# Autodesk Inventor assembly: 2013 Drive in a Day Frame
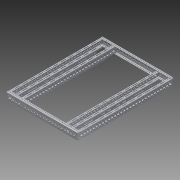
[picture p0: Inventor's stored thumbnail of the model, 180x180]
Saved by Autodesk Inventor 2013 (Build 170138000, 138)
## iProperties
Created: 2013-05-24
Part Number: 2013 Drive in a Day Frame
Document SubType Name: Assembly
Designer: natsidhu
Author: natsidhu
## Documents named in this file (3)
- \\lmss\students\Robotics\CAD Files\COTS Parts\Kit Frame - VexPro\2013 Drive in a Day Frame.iam
- \\lmss\students\Robotics\CAD Files\COTS Parts\Kit Frame - VexPro\217-2593-002 Rev3 - Front Rail.ipt
- \\lmss\students\Robotics\CAD Files\COTS Parts\Kit Frame - VexPro\217-2593-001 Rev2 - Side Rail.ipt
## Components (6 placed, 2 different names)
1. 217-2593-002 Rev3 - Front Rail:1 — Flush:1, Mate:2, Flush:2, Mate:9, Flush:5, Mate:11, Flush:6
2. 217-2593-001 Rev2 - Side Rail:1 — Mate:1, Mate:2, Mate:4, Mate:5, Mate:7, Flush:2, Flush:3
3. 217-2593-001 Rev2 - Side Rail:2 — Mate:8, Mate:9, Flush:4
4. 217-2593-002 Rev3 - Front Rail:2 — Mate:5, Mate:7, Flush:3, Mate:8, Flush:4, Mate:12
5. 217-2593-001 Rev2 - Side Rail:3 — Flush:6, Flush:7, Mate:12
6. 217-2593-001 Rev2 - Side Rail:4 — Flush:5, Mate:10, Mate:11
## Relationships (17: Mate 10, Flush 7)
- Flush:1: 217-2593-002 Rev3 - Front Rail:1
- Mate:1: 217-2593-001 Rev2 - Side Rail:1
- Mate:2: 217-2593-002 Rev3 - Front Rail:1 ↔ 217-2593-001 Rev2 - Side Rail:1
- Mate:4 (44.1198 mm): 217-2593-001 Rev2 - Side Rail:1
- Mate:5: 217-2593-001 Rev2 - Side Rail:1 ↔ 217-2593-002 Rev3 - Front Rail:2
- Mate:7: 217-2593-001 Rev2 - Side Rail:1 ↔ 217-2593-002 Rev3 - Front Rail:2
- Flush:2: 217-2593-002 Rev3 - Front Rail:1 ↔ 217-2593-001 Rev2 - Side Rail:1
- Flush:3: 217-2593-001 Rev2 - Side Rail:1 ↔ 217-2593-002 Rev3 - Front Rail:2
- Mate:8: 217-2593-001 Rev2 - Side Rail:2 ↔ 217-2593-002 Rev3 - Front Rail:2
- Mate:9: 217-2593-002 Rev3 - Front Rail:1 ↔ 217-2593-001 Rev2 - Side Rail:2
- Flush:4: 217-2593-001 Rev2 - Side Rail:2 ↔ 217-2593-002 Rev3 - Front Rail:2
- Flush:5: 217-2593-002 Rev3 - Front Rail:1 ↔ 217-2593-001 Rev2 - Side Rail:4
- Mate:10: 217-2593-001 Rev2 - Side Rail:4
- Mate:11: 217-2593-002 Rev3 - Front Rail:1 ↔ 217-2593-001 Rev2 - Side Rail:4
- Flush:6: 217-2593-002 Rev3 - Front Rail:1 ↔ 217-2593-001 Rev2 - Side Rail:3
- Flush:7: 217-2593-001 Rev2 - Side Rail:3
- Mate:12: 217-2593-002 Rev3 - Front Rail:2 ↔ 217-2593-001 Rev2 - Side Rail:3
